# Autodesk Inventor assembly: YAxis_Carriage
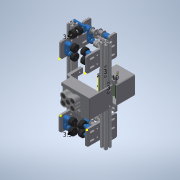
[picture p0: Inventor's stored thumbnail of the model, 180x180]
Saved by Autodesk Inventor 2021 (Build 250183000, 183)
## iProperties
Created: 2021-02-02
Part Number: YAxis_Carriage
Document SubType Name: Assembly
Designer: Jorian Brusind
Author: Jorian Brusind
## Documents named in this file (17)
- C:\Users\Jorian Bruslind\Documents\GitHub\PersonalProjects\HyperRail\Inventor Files\YAxis_Carriage.iam
- C:\Users\Jorian Bruslind\Documents\GitHub\PersonalProjects\Inventor Projects\Useful models\8020_Sets\IPT_20_Series\IPT_20_Series\20-2020_300mm.ipt
- C:\Users\Jorian Bruslind\Documents\GitHub\PersonalProjects\Inventor Projects\Useful models\NEMA_Steppers\nema-17-stepper-motor-with-v2-damper-1.snapshot.3\Nema 17  Stepper Motor length 34mm.ipt
- C:\Users\Jorian Bruslind\Documents\GitHub\PersonalProjects\HyperRail\Inventor Files\SmallBelt_Pulley.ipt
- C:\Users\Jorian Bruslind\Documents\GitHub\PersonalProjects\Inventor Projects\Useful models\Metric bolt\Bolt M3 30mm.ipt
- C:\Users\Jorian Bruslind\Documents\GitHub\PersonalProjects\HyperRail\Inventor Files\small_belt_loop.ipt
- C:\Users\Jorian Bruslind\Documents\GitHub\PersonalProjects\HyperRail\PCB Files\Integrated Stepper Motor Driver\ExportSTEP\Main.iam
- C:\Users\Jorian Bruslind\Documents\GitHub\PersonalProjects\HyperRail\Inventor Files\rededge-micasense-1.snapshot.3\PND_CAM_MSRE.ipt
- C:\Users\Jorian Bruslind\Documents\GitHub\PersonalProjects\HyperRail\Inventor Files\Camera_Mount.ipt
- C:\Users\Jorian Bruslind\Documents\GitHub\PersonalProjects\HyperRail\Inventor Files\F623ZZ v2.iam
- C:\Users\Jorian Bruslind\Documents\GitHub\PersonalProjects\HyperRail\Inventor Files\6mm_Spacer.ipt
- C:\Users\Jorian Bruslind\Documents\GitHub\PersonalProjects\HyperRail\Inventor Files\NEMA17_Shroud.ipt
- C:\Users\Jorian Bruslind\Documents\GitHub\PersonalProjects\HyperRail\Inventor Files\Buffer.iam
- C:\Users\Jorian Bruslind\Documents\GitHub\PersonalProjects\HyperRail\Inventor Files\X_Carriage_V2_0.iam
- C:\Users\Jorian Bruslind\Documents\GitHub\PersonalProjects\HyperRail\Inventor Files\X_CarriageR_V2_0.iam
- C:\Users\Jorian Bruslind\Documents\GitHub\PersonalProjects\HyperRail\Inventor Files\X_CarriageR_V2_1.iam
- C:\Users\Jorian Bruslind\Documents\GitHub\PersonalProjects\HyperRail\Inventor Files\X_Carriage_V2_1.iam
## Components (31 placed, 16 different names)
1. 20-2020_300mm:1 — Flush:25, Mate:59, Flush:27, Mate:106, Flush:66, Flush:67, Mate:140, Mate:141, Flush:70, Flush:71
2. Nema 17  Stepper Motor length 34mm:1 — Mate:13, Mate:14, Mate:36, Mate:42, Flush:14, Flush:15
3. SmallBelt_Pulley:1 — Mate:13, Mate:14, Mate:37, Flush:33, Flush:34
4. Bolt M3 30mm:1 — Mate:65, Mate:66, Flush:35, Mate:94
5. Bolt M3 30mm:2 — Mate:38, Mate:63, Mate:64, Flush:36, Mate:95
6. small_belt_loop:1 — Mate:36, Mate:37, Mate:38
7. Main:1 [sub-assembly] — Mate:42, Flush:14, Flush:15, Mate:105
8. 20-2020_300mm:2 — Flush:25, Flush:26, Flush:27, Mate:108, Mate:109, Flush:50, Flush:52, Flush:56, Mate:121, Mate:124, Mate:126
9. PND_CAM_MSRE:1 — Mate:47, Mate:48, Mate:49
10. Camera_Mount:1 — Mate:47, Mate:48, Mate:49, Mate:59, Flush:26
11. F623ZZ v2:1 [sub-assembly] — Mate:65, Mate:67, Flush:34
12. F623ZZ v2:2 [sub-assembly] — Mate:66, Mate:67, Mate:99
13. F623ZZ v2:3 [sub-assembly] — Mate:63, Mate:68, Flush:33
14. F623ZZ v2:4 [sub-assembly] — Mate:64, Mate:68, Mate:96
15. Bolt M3 30mm:3 — Flush:35, Flush:36, Flush:37, Mate:88
16. F623ZZ v2:5 [sub-assembly]
17. F623ZZ v2:6 [sub-assembly]
18. Bolt M3 30mm:4 — Flush:37, Mate:93
19. F623ZZ v2:7 [sub-assembly]
20. F623ZZ v2:8 [sub-assembly] — Mate:97
21. 6mm_Spacer:1 — Mate:88
22. 6mm_Spacer:6 — Mate:93, Mate:97
23. 6mm_Spacer:8 — Mate:95, Mate:96
24. 6mm_Spacer:10 — Mate:94, Mate:99
25. NEMA17_Shroud:1 — Mate:105, Mate:106
26. Buffer:1 [sub-assembly] — Mate:108, Flush:52, Flush:56
27. Buffer:3 [sub-assembly] — Mate:109, Flush:50, Mate:125
28. X_Carriage_V2_0:1 [sub-assembly] — Mate:124, Mate:125, Mate:143, Mate:144
29. X_CarriageR_V2_0:2 [sub-assembly] — Mate:126, Flush:69, Mate:142
30. X_CarriageR_V2_1:1 [sub-assembly] — Mate:140, Flush:68, Flush:69, Flush:70, Mate:143, Mate:144
31. X_Carriage_V2_1:1 [sub-assembly] — Mate:141, Flush:68, Flush:71, Mate:142
## Relationships (61: Mate 42, Flush 19)
- Mate:13: Nema 17  Stepper Motor length 34mm:1 ↔ SmallBelt_Pulley:1
- Mate:14: Nema 17  Stepper Motor length 34mm:1 ↔ SmallBelt_Pulley:1
- Mate:36: Nema 17  Stepper Motor length 34mm:1 ↔ small_belt_loop:1
- Mate:37 (2 mm): SmallBelt_Pulley:1 ↔ small_belt_loop:1
- Mate:38: Bolt M3 30mm:2 ↔ small_belt_loop:1
- Mate:42 (5 mm): Nema 17  Stepper Motor length 34mm:1 ↔ Main:1
- Flush:14: Nema 17  Stepper Motor length 34mm:1 ↔ Main:1
- Flush:15: Nema 17  Stepper Motor length 34mm:1 ↔ Main:1
- Mate:47: PND_CAM_MSRE:1 ↔ Camera_Mount:1
- Mate:48: PND_CAM_MSRE:1 ↔ Camera_Mount:1
- Mate:49: PND_CAM_MSRE:1 ↔ Camera_Mount:1
- Flush:25: 20-2020_300mm:1 ↔ 20-2020_300mm:2
- Mate:59: 20-2020_300mm:1 ↔ Camera_Mount:1
- Flush:26: 20-2020_300mm:2 ↔ Camera_Mount:1
- Flush:27: 20-2020_300mm:1 ↔ 20-2020_300mm:2
- Mate:63: Bolt M3 30mm:2 ↔ F623ZZ v2:3
- Mate:64: Bolt M3 30mm:2 ↔ F623ZZ v2:4
- Mate:65: Bolt M3 30mm:1 ↔ F623ZZ v2:1
- Mate:66: Bolt M3 30mm:1 ↔ F623ZZ v2:2
- Mate:67: F623ZZ v2:1 ↔ F623ZZ v2:2
- Mate:68: F623ZZ v2:3 ↔ F623ZZ v2:4
- Flush:33 (2 mm): SmallBelt_Pulley:1 ↔ F623ZZ v2:3
- Flush:34 (2 mm): SmallBelt_Pulley:1 ↔ F623ZZ v2:1
- [Mate]: Bolt M3 30mm:3 ↔ F623ZZ v2:5
- [Mate]: Bolt M3 30mm:3 ↔ F623ZZ v2:6
- [Mate]: F623ZZ v2:5 ↔ F623ZZ v2:6
- [Mate]: Bolt M3 30mm:4 ↔ F623ZZ v2:7
- [Mate]: Bolt M3 30mm:4 ↔ F623ZZ v2:8
- [Mate]: F623ZZ v2:7 ↔ F623ZZ v2:8
- Flush:35: Bolt M3 30mm:1 ↔ Bolt M3 30mm:3
- Flush:36: Bolt M3 30mm:2 ↔ Bolt M3 30mm:3
- Flush:37: Bolt M3 30mm:3 ↔ Bolt M3 30mm:4
- Mate:88: Bolt M3 30mm:3 ↔ 6mm_Spacer:1
- Mate:93: Bolt M3 30mm:4 ↔ 6mm_Spacer:6
- Mate:94: Bolt M3 30mm:1 ↔ 6mm_Spacer:10
- Mate:95: Bolt M3 30mm:2 ↔ 6mm_Spacer:8
- Mate:96: F623ZZ v2:4 ↔ 6mm_Spacer:8
- Mate:97: F623ZZ v2:8 ↔ 6mm_Spacer:6
- Mate:99: F623ZZ v2:2 ↔ 6mm_Spacer:10
- Mate:105: Main:1 ↔ NEMA17_Shroud:1
- Mate:106: 20-2020_300mm:1 ↔ NEMA17_Shroud:1
- Mate:108: 20-2020_300mm:2 ↔ Buffer:1
- Mate:109: 20-2020_300mm:2 ↔ Buffer:3
- Flush:50: 20-2020_300mm:2 ↔ Buffer:3
- Flush:52: 20-2020_300mm:2 ↔ Buffer:1
- Flush:56: 20-2020_300mm:2 ↔ Buffer:1
- Mate:121: 20-2020_300mm:2
- Flush:66: 20-2020_300mm:1
- Flush:67: 20-2020_300mm:1
- Mate:124: 20-2020_300mm:2 ↔ X_Carriage_V2_0:1
- Mate:125 (4 mm): Buffer:3 ↔ X_Carriage_V2_0:1
- Mate:126: 20-2020_300mm:2 ↔ X_CarriageR_V2_0:2
- Mate:140: 20-2020_300mm:1 ↔ X_CarriageR_V2_1:1
- Mate:141: 20-2020_300mm:1 ↔ X_Carriage_V2_1:1
- Flush:68: X_CarriageR_V2_1:1 ↔ X_Carriage_V2_1:1
- Flush:69: X_CarriageR_V2_0:2 ↔ X_CarriageR_V2_1:1
- Flush:70: 20-2020_300mm:1 ↔ X_CarriageR_V2_1:1
- Flush:71: 20-2020_300mm:1 ↔ X_Carriage_V2_1:1
- Mate:142: X_CarriageR_V2_0:2 ↔ X_Carriage_V2_1:1
- Mate:143: X_Carriage_V2_0:1 ↔ X_CarriageR_V2_1:1
- Mate:144 (10 mm): X_Carriage_V2_0:1 ↔ X_CarriageR_V2_1:1
## Named parameters: d133_d125 = 0 mm, d134_d126 = 0 mm, d135_d130 = 0 mm, d136_d125 = 0 mm, d137_d126 = 0 mm, d138_d130 = 0 mm
